# Autodesk Inventor assembly: Portal Companion Cube
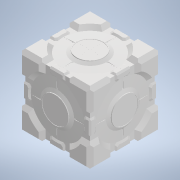
[picture p0: Inventor's stored thumbnail of the model, 180x180]
Saved by Autodesk Inventor 2020 (Build 240168000, 168)
## iProperties
Created: 2020-01-12
Part Number: Portal Companion Cube
Document SubType Name: Assembly
Designer: maple
Author: maple
## Documents named in this file (3)
- C:\Users\maple\Desktop\Portal Companion Cube.iam
- C:\Users\maple\Desktop\Portal Companion Cube.ipt
- C:\Users\maple\Desktop\Portal Companion Cube_MIR.ipt
## Components (8 placed, 2 different names)
1. Portal Companion Cube:1
2. Portal Companion Cube:2
3. Portal Companion Cube:3
4. Portal Companion Cube:4
5. Portal Companion Cube_MIR:1
6. Portal Companion Cube_MIR:2
7. Portal Companion Cube_MIR:3
8. Portal Companion Cube_MIR:4
## Component patterns: (4 elements, first: Portal Companion Cube:1), (4 elements, first: Portal Companion Cube_MIR:1)
